# Autodesk Inventor assembly: winch
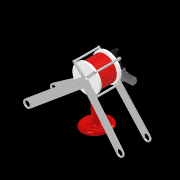
[picture p0: Inventor's stored thumbnail of the model, 180x180]
Saved by Autodesk Inventor 2020.2 (Build 242310000, 310)
## iProperties
Created: 2020-03-23
Part Number: winch
Document SubType Name: Assembly
Designer: agmle
Mass: 6591.26 g
Surface Area: 4788.33 cm^2
Volume: 2717.61 cm^3
Density: 2.42539 g/cm^3
Author: agmle
## Documents named in this file (19)
- D:\syncthing\rwsir-rc7py\projects\CreekFleet\CreekFleet_AutoBuoy\Mechanical CAD\station-keeping\winch.iam
- D:\syncthing\rwsir-rc7py\projects\CreekFleet\CreekFleet_AutoBuoy\Mechanical CAD\station-keeping\Window Motor Right.ipt
- D:\syncthing\rwsir-rc7py\projects\CreekFleet\CreekFleet_AutoBuoy\Mechanical CAD\station-keeping\winch_drum.ipt
- D:\syncthing\rwsir-rc7py\projects\CreekFleet\CreekFleet_AutoBuoy\Mechanical CAD\propulsion\bearing\6138k63.iam
- D:\syncthing\rwsir-rc7py\projects\CreekFleet\CreekFleet_AutoBuoy\Mechanical CAD\station-keeping\shaft.ipt
- D:\syncthing\rwsir-rc7py\projects\CreekFleet\CreekFleet_AutoBuoy\Mechanical CAD\station-keeping\motor_support.ipt
- D:\syncthing\rwsir-rc7py\Inventor\Content Center Files\R2020\en-US\ANSI B18.3.1M(6)\ANSI B18.3.1M - M5x0.8 x 40(1).ipt
- D:\syncthing\rwsir-rc7py\Inventor\Content Center Files\R2020\en-US\ANSI B18.3.1M(6)\ANSI B18.3.1M - M5x0.8 x 30(1).ipt
- D:\syncthing\rwsir-rc7py\projects\CreekFleet\CreekFleet_AutoBuoy\Mechanical CAD\station-keeping\strut.ipt
- D:\syncthing\rwsir-rc7py\Inventor\Content Center Files\R2020\en-US\ASME ANSI B18.3.5M(1)\ASME_ANSI B18.3.5M - M5x14(1).ipt
- D:\syncthing\rwsir-rc7py\projects\CreekFleet\CreekFleet_AutoBuoy\Mechanical CAD\station-keeping\winch_support.ipt
- D:\syncthing\rwsir-rc7py\projects\CreekFleet\CreekFleet_AutoBuoy\Mechanical CAD\station-keeping\anchor.ipt
- D:\syncthing\rwsir-rc7py\Inventor\Content Center Files\R2020\en-US\ANSI B18.22.1\ANSI B18.22.1 - No. 5 - narrow - Type B.ipt
- D:\syncthing\rwsir-rc7py\projects\CreekFleet\CreekFleet_AutoBuoy\Mechanical CAD\station-keeping\anchor_line.ipt
- D:\syncthing\rwsir-rc7py\Inventor\Content Center Files\R2020\en-US\ASME ANSI B18.3.5M(1)\ASME_ANSI B18.3.5M - M3x10(1).ipt
- D:\syncthing\rwsir-rc7py\projects\CreekFleet\CreekFleet_AutoBuoy\Mechanical CAD\station-keeping\winch_support_port_forward.ipt
- D:\syncthing\rwsir-rc7py\projects\CreekFleet\CreekFleet_AutoBuoy\Mechanical CAD\station-keeping\winch_support_port_aft.ipt
- D:\syncthing\rwsir-rc7py\projects\CreekFleet\CreekFleet_AutoBuoy\Mechanical CAD\station-keeping\winch_support_starboard_forward.ipt
- D:\syncthing\rwsir-rc7py\projects\CreekFleet\CreekFleet_AutoBuoy\Mechanical CAD\station-keeping\winch_support_starboard_aft.ipt
## Components (38 placed, 18 different names)
1. winch_support_port_forward:1 — Insert:43, Insert:44, Insert:45, Insert:46, Insert:47
2. winch_support_port_aft:1 — Insert:48, Insert:49, Insert:50, Insert:51, Insert:52
3. winch_support_starboard_forward:1 — Insert:53, Insert:54, Insert:59, Insert:60
4. winch_support_starboard_aft:1 — Insert:57, Insert:58, Insert:61, Insert:62
5. Plain Washer (Inch) No. 5 - narrow - Type B:1 — Insert:25, Insert:26
6. winch_drum:1 — Insert:25, Mate:2, Mate:5
7. 6138k63:1 [sub-assembly] — Insert:3, Insert:26, Insert:42
8. shaft:1 — Insert:3
9. Window Motor Right:1 — Insert:6, Insert:7, Insert:8, Insert:9, Insert:10
10. Forged Socket Head Cap Screw - Metric M5x0.8 x 40:1 — Insert:8
11. Forged Socket Head Cap Screw - Metric M5x0.8 x 30:1 — Insert:7
12. Forged Socket Head Cap Screw - Metric M5x0.8 x 30:2 — Insert:6
13. motor_support:1 — Insert:9, Insert:10, Insert:11, Insert:12, Insert:13, Insert:14, Insert:15, Insert:16, Insert:17, Insert:18, Insert:53, Insert:54, Insert:57, Insert:58
14. strut:1 — Insert:12, Insert:19
15. strut:2 — Insert:11, Insert:20
16. strut:3 — Insert:13
17. strut:4 — Insert:14
18. Forged Hexagon Socket Flat Countersunk Head Cap Screws - Metric M5x14:1 — Insert:15
19. Forged Hexagon Socket Flat Countersunk Head Cap Screws - Metric M5x14:2 — Insert:17
20. Forged Hexagon Socket Flat Countersunk Head Cap Screws - Metric M5x14:3 — Insert:16
21. Forged Hexagon Socket Flat Countersunk Head Cap Screws - Metric M5x14:4 — Insert:18
22. winch_support:1 — Insert:19, Insert:20, Insert:21, Insert:22, Insert:23, Insert:24, Insert:42, Insert:43, Insert:44, Insert:48, Insert:49
23. Forged Hexagon Socket Flat Countersunk Head Cap Screws - Metric M5x14:5 — Insert:24
24. Forged Hexagon Socket Flat Countersunk Head Cap Screws - Metric M5x14:6 — Insert:23
25. Forged Hexagon Socket Flat Countersunk Head Cap Screws - Metric M5x14:7 — Insert:22
26. Forged Hexagon Socket Flat Countersunk Head Cap Screws - Metric M5x14:8 — Insert:21
27. anchor:1 — Mate:3, Mate:4
28. anchor_line:1 — Mate:2, Mate:3, Mate:4, Mate:5
29. Forged Hexagon Socket Flat Countersunk Head Cap Screws - Metric M3x10:7 — Insert:61
30. Forged Hexagon Socket Flat Countersunk Head Cap Screws - Metric M3x10:8 — Insert:62
31. Forged Hexagon Socket Flat Countersunk Head Cap Screws - Metric M3x10:10 — Insert:59
32. Forged Hexagon Socket Flat Countersunk Head Cap Screws - Metric M3x10:11 — Insert:60
33. Forged Hexagon Socket Flat Countersunk Head Cap Screws - Metric M3x10:1 — Insert:52
34. Forged Hexagon Socket Flat Countersunk Head Cap Screws - Metric M3x10:2 — Insert:51
35. Forged Hexagon Socket Flat Countersunk Head Cap Screws - Metric M3x10:3 — Insert:47
36. Forged Hexagon Socket Flat Countersunk Head Cap Screws - Metric M3x10:4 — Insert:46
37. Forged Hexagon Socket Flat Countersunk Head Cap Screws - Metric M3x10:5 — Insert:50
38. Forged Hexagon Socket Flat Countersunk Head Cap Screws - Metric M3x10:6 — Insert:45
## Relationships (45: Insert 41, Mate 4)
- Insert:3: 6138k63:1 ↔ shaft:1
- Insert:6: Window Motor Right:1 ↔ Forged Socket Head Cap Screw - Metric M5x0.8 x 30:2
- Insert:7: Window Motor Right:1 ↔ Forged Socket Head Cap Screw - Metric M5x0.8 x 30:1
- Insert:8: Window Motor Right:1 ↔ Forged Socket Head Cap Screw - Metric M5x0.8 x 40:1
- Insert:9: Window Motor Right:1 ↔ motor_support:1
- Insert:10: Window Motor Right:1 ↔ motor_support:1
- Insert:11: motor_support:1 ↔ strut:2
- Insert:12: motor_support:1 ↔ strut:1
- Insert:13: motor_support:1 ↔ strut:3
- Insert:14: motor_support:1 ↔ strut:4
- Insert:15: motor_support:1 ↔ Forged Hexagon Socket Flat Countersunk Head Cap Screws - Metric M5x14:1
- Insert:16: motor_support:1 ↔ Forged Hexagon Socket Flat Countersunk Head Cap Screws - Metric M5x14:3
- Insert:17: motor_support:1 ↔ Forged Hexagon Socket Flat Countersunk Head Cap Screws - Metric M5x14:2
- Insert:18: motor_support:1 ↔ Forged Hexagon Socket Flat Countersunk Head Cap Screws - Metric M5x14:4
- Insert:19: strut:1 ↔ winch_support:1
- Insert:20: strut:2 ↔ winch_support:1
- Insert:21: winch_support:1 ↔ Forged Hexagon Socket Flat Countersunk Head Cap Screws - Metric M5x14:8
- Insert:22: winch_support:1 ↔ Forged Hexagon Socket Flat Countersunk Head Cap Screws - Metric M5x14:7
- Insert:23: winch_support:1 ↔ Forged Hexagon Socket Flat Countersunk Head Cap Screws - Metric M5x14:6
- Insert:24: winch_support:1 ↔ Forged Hexagon Socket Flat Countersunk Head Cap Screws - Metric M5x14:5
- Insert:25: Plain Washer (Inch) No. 5 - narrow - Type B:1 ↔ winch_drum:1
- Insert:26: Plain Washer (Inch) No. 5 - narrow - Type B:1 ↔ 6138k63:1
- Mate:2: winch_drum:1 ↔ anchor_line:1
- Mate:3: anchor:1 ↔ anchor_line:1
- Mate:4: anchor:1 ↔ anchor_line:1
- Mate:5: winch_drum:1 ↔ anchor_line:1
- Insert:42: 6138k63:1 ↔ winch_support:1
- Insert:43: winch_support_port_forward:1 ↔ winch_support:1
- Insert:44: winch_support_port_forward:1 ↔ winch_support:1
- Insert:45: winch_support_port_forward:1 ↔ Forged Hexagon Socket Flat Countersunk Head Cap Screws - Metric M3x10:6
- Insert:46: winch_support_port_forward:1 ↔ Forged Hexagon Socket Flat Countersunk Head Cap Screws - Metric M3x10:4
- Insert:47: winch_support_port_forward:1 ↔ Forged Hexagon Socket Flat Countersunk Head Cap Screws - Metric M3x10:3
- Insert:48: winch_support_port_aft:1 ↔ winch_support:1
- Insert:49: winch_support_port_aft:1 ↔ winch_support:1
- Insert:50: winch_support_port_aft:1 ↔ Forged Hexagon Socket Flat Countersunk Head Cap Screws - Metric M3x10:5
- Insert:51: winch_support_port_aft:1 ↔ Forged Hexagon Socket Flat Countersunk Head Cap Screws - Metric M3x10:2
- Insert:52: winch_support_port_aft:1 ↔ Forged Hexagon Socket Flat Countersunk Head Cap Screws - Metric M3x10:1
- Insert:53: winch_support_starboard_forward:1 ↔ motor_support:1
- Insert:54: winch_support_starboard_forward:1 ↔ motor_support:1
- Insert:57: winch_support_starboard_aft:1 ↔ motor_support:1
- Insert:58: winch_support_starboard_aft:1 ↔ motor_support:1
- Insert:59: winch_support_starboard_forward:1 ↔ Forged Hexagon Socket Flat Countersunk Head Cap Screws - Metric M3x10:10
- Insert:60: winch_support_starboard_forward:1 ↔ Forged Hexagon Socket Flat Countersunk Head Cap Screws - Metric M3x10:11
- Insert:61: winch_support_starboard_aft:1 ↔ Forged Hexagon Socket Flat Countersunk Head Cap Screws - Metric M3x10:7
- Insert:62: winch_support_starboard_aft:1 ↔ Forged Hexagon Socket Flat Countersunk Head Cap Screws - Metric M3x10:8
